# Autodesk Inventor assembly: noga_pre
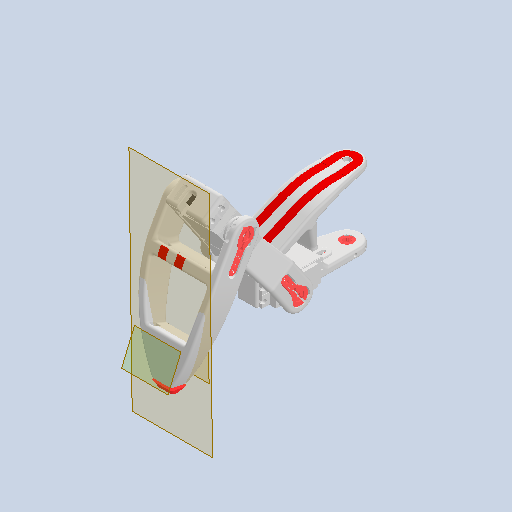
[picture p0: Inventor's stored thumbnail of the model, 512x512]
Saved by Autodesk Inventor 2023.4 (Build 274418000, 418)
## iProperties
Created: 2024-06-27
Part Number: noga_pre
Document SubType Name: Assembly
Designer: kamil
Author: kamil
## Documents named in this file (11)
- E:\PROJECTS_REPOS\Robal-2.0\mechanics\noga_pre.iam
- E:\PROJECTS_REPOS\Robal-2.0\mechanics\Standard-Servo.ipt
- E:\PROJECTS_REPOS\Robal-2.0\mechanics\czlon2_pre.ipt
- E:\PROJECTS_REPOS\Robal-2.0\mechanics\czlon3_pre.ipt
- E:\PROJECTS_REPOS\Robal-2.0\mechanics\SERVO ARM HORN 25T ALUMINIUM\SERVO ARM HORN 25T ALUMINIUM.ipt
- E:\PROJECTS_REPOS\Robal-2.0\mechanics\czlon_2_wciecie_1.ipt
- E:\PROJECTS_REPOS\Robal-2.0\mechanics\czlon_2_wciecie_2.ipt
- E:\PROJECTS_REPOS\Robal-2.0\mechanics\czlon_2_wciecie_3.ipt
- E:\PROJECTS_REPOS\Robal-2.0\mechanics\czlon_3_wciecie_1.ipt
- E:\PROJECTS_REPOS\Robal-2.0\mechanics\czlon_3_wciecie_2.ipt
- E:\PROJECTS_REPOS\Robal-2.0\mechanics\czlon_4_zloz.iam
## Components (13 placed, 10 different names)
1. Standard-Servo:1 — Zestawiające:9, Zestawiające:11, Mate:24, Mate:25, Mate:26
2. czlon2_pre:1 — Zestawiające:9, Zestawiające:11, Angle:1, Mate:26, Mate:32, Mate:33, Mate:35, Mate:36, Mate:37, Mate:38, Mate:39, Zestawiające:48, Zestawiające:49
3. czlon3_pre:1 — Zestawiające:48, Zestawiające:49, Zestawiające:50, Zestawiające:51, Zestawiające:52, Zestawiające:53, Zestawiające:54, Zestawiające:55, Zestawiające:56, Zestawiające:57, Kątowe:6, Zestawiające:58, Zestawiające:59
4. Standard-Servo:3 — Mate:46, Mate:47, Zestawiające:58, Zestawiające:59
5. SERVO ARM HORN 25T ALUMINIUM:1 — Angle:1
6. SERVO ARM HORN 25T ALUMINIUM:2 — Mate:24, Mate:25, Flush:5, Kątowe:6
7. czlon_2_wciecie_1:1 — Mate:32, Mate:33, Mate:37, Angle:3
8. czlon_2_wciecie_2:1 — Mate:35, Mate:36
9. czlon_2_wciecie_3:1 — Mate:38, Mate:39, Angle:3
10. czlon_3_wciecie_1:1 — Zestawiające:50, Zestawiające:51, Zestawiające:52
11. czlon_3_wciecie_2:1 — Zestawiające:53, Zestawiające:55, Zestawiające:56
12. SERVO ARM HORN 25T ALUMINIUM:3 — Flush:5, Mate:46, Angle:5, Kątowe:7
13. czlon_4_zloz:1 [sub-assembly] — Mate:47, Angle:5, Zestawiające:54, Zestawiające:57, Kątowe:7
## Relationships (32: Mate 26, Angle 5, Flush 1)
- Zestawiające:9 [Mate] (1 mm): Standard-Servo:1 ↔ czlon2_pre:1
- Zestawiające:11 [Mate]: Standard-Servo:1 ↔ czlon2_pre:1
- Angle:1 (0 deg): czlon2_pre:1 ↔ SERVO ARM HORN 25T ALUMINIUM:1
- Mate:24: Standard-Servo:1 ↔ SERVO ARM HORN 25T ALUMINIUM:2
- Mate:25: Standard-Servo:1 ↔ SERVO ARM HORN 25T ALUMINIUM:2
- Mate:26: Standard-Servo:1 ↔ czlon2_pre:1
- Mate:32: czlon2_pre:1 ↔ czlon_2_wciecie_1:1
- Mate:33: czlon2_pre:1 ↔ czlon_2_wciecie_1:1
- Mate:35: czlon2_pre:1 ↔ czlon_2_wciecie_2:1
- Mate:36: czlon2_pre:1 ↔ czlon_2_wciecie_2:1
- Mate:37 (0.1 mm): czlon2_pre:1 ↔ czlon_2_wciecie_1:1
- Mate:38: czlon2_pre:1 ↔ czlon_2_wciecie_3:1
- Mate:39: czlon2_pre:1 ↔ czlon_2_wciecie_3:1
- Angle:3 (180 deg): czlon_2_wciecie_1:1 ↔ czlon_2_wciecie_3:1
- Flush:5: SERVO ARM HORN 25T ALUMINIUM:2 ↔ SERVO ARM HORN 25T ALUMINIUM:3
- Mate:46: Standard-Servo:3 ↔ SERVO ARM HORN 25T ALUMINIUM:3
- Mate:47 (0.1 mm): Standard-Servo:3 ↔ czlon_4_zloz:1
- Angle:5 (180 deg): SERVO ARM HORN 25T ALUMINIUM:3 ↔ czlon_4_zloz:1
- Zestawiające:48 [Mate] (2 mm): czlon2_pre:1 ↔ czlon3_pre:1
- Zestawiające:49 [Mate]: czlon2_pre:1 ↔ czlon3_pre:1
- Zestawiające:50 [Mate]: czlon3_pre:1 ↔ czlon_3_wciecie_1:1
- Zestawiające:51 [Mate]: czlon3_pre:1 ↔ czlon_3_wciecie_1:1
- Zestawiające:52 [Mate]: czlon3_pre:1 ↔ czlon_3_wciecie_1:1
- Zestawiające:53 [Mate]: czlon3_pre:1 ↔ czlon_3_wciecie_2:1
- Zestawiające:54 [Mate]: czlon3_pre:1 ↔ czlon_4_zloz:1
- Zestawiające:55 [Mate]: czlon3_pre:1 ↔ czlon_3_wciecie_2:1
- Zestawiające:56 [Mate]: czlon3_pre:1 ↔ czlon_3_wciecie_2:1
- Zestawiające:57 [Mate] (2 mm): czlon3_pre:1 ↔ czlon_4_zloz:1
- Kątowe:6 [Angle] (180 deg): czlon3_pre:1 ↔ SERVO ARM HORN 25T ALUMINIUM:2
- Kątowe:7 [Angle] (180 deg): SERVO ARM HORN 25T ALUMINIUM:3 ↔ czlon_4_zloz:1
- Zestawiające:58 [Mate]: czlon3_pre:1 ↔ Standard-Servo:3
- Zestawiające:59 [Mate]: czlon3_pre:1 ↔ Standard-Servo:3
